# Autodesk Inventor assembly: 788640001
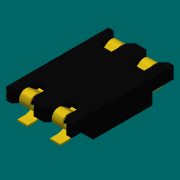
[picture p0: Inventor's stored thumbnail of the model, 180x180]
Saved by Autodesk Inventor 2016 (Build 200138000, 138)
## iProperties
Created: 2015-10-16
Part Number: 788640001
Document SubType Name: Assembly
Designer: Sawaiz
Author: Sawaiz
## Documents named in this file (2)
- C:\Users\Sawaiz\OneDrive\projects\mppcSensorInterface\cad\electronics\788640001\788640001.iam
- C:\Users\Sawaiz\OneDrive\projects\mppcSensorInterface\cad\electronics\788640001\788640001.ipt
## Components (2 placed, 1 different names)
1. 788640001:1 — Mate:1, Flush:1, Flush:2
2. 788640001:2 — Mate:1, Flush:1, Flush:2
## Relationships (3: Flush 2, Mate 1)
- Mate:1: 788640001:1 ↔ 788640001:2
- Flush:1: 788640001:1 ↔ 788640001:2
- Flush:2: 788640001:1 ↔ 788640001:2
